# Autodesk Inventor assembly: RCUAssy
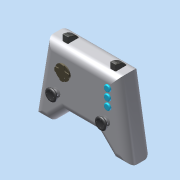
[picture p0: Inventor's stored thumbnail of the model, 180x180]
Saved by Autodesk Inventor 2011 SP1 (Build 150282100, 282)
## iProperties
Created: 2011-08-15
Part Number: RCUAssy
Document SubType Name: Assembly
Designer: dgitz
Author: dgitz
## Documents named in this file (6)
- C:\Dropbox\ICARUS\Remote Control Unit (RCU)\RCU v2\Design\RCUv2-2\RCUAssy.iam
- C:\Dropbox\ICARUS\Remote Control Unit (RCU)\RCU v2\Design\RCUv2-2\RUCBase.ipt
- C:\Dropbox\ICARUS\Remote Control Unit (RCU)\RCU v2\Design\Library\Trigger.ipt
- C:\Dropbox\ICARUS\Remote Control Unit (RCU)\RCU v2\Design\Imported Components\User Library-Joystick_Asm_Left\Assembly3.iam
- C:\Dropbox\ICARUS\Remote Control Unit (RCU)\RCU v2\Design\Library\Xbox360Button.ipt
- C:\Dropbox\ICARUS\Remote Control Unit (RCU)\RCU v2\Design\Library\XBox360DirectionalPad.ipt
## Components (9 placed, 5 different names)
1. RUCBase:1 — Mate:1, Mate:2, Mate:4, Mate:8, Mate:9
2. Trigger:1 — Insert:1, Flush:4, Mate:9
3. Trigger:2 — Insert:1, Flush:4
4. Assembly3:1 [sub-assembly] — Mate:1, Flush:1, Mate:3
5. Assembly3:2 [sub-assembly] — Mate:2, Flush:1, Mate:3
6. XBox360DirectionalPad:1 — Mate:4, Mate:5
7. Xbox360Button:2 — Mate:6, Mate:7, Flush:2, Flush:3
8. Xbox360Button:3 — Mate:7, Flush:3, Mate:8
9. Xbox360Button:4 — Mate:6, Flush:2
## Relationships (14: Mate 9, Flush 4, Insert 1)
- Mate:1 (-6.35 mm): RUCBase:1 ↔ Assembly3:1
- Mate:2 (-6.35 mm): RUCBase:1 ↔ Assembly3:2
- Flush:1: Assembly3:1 ↔ Assembly3:2
- Mate:3 (63.5 mm): Assembly3:1 ↔ Assembly3:2
- Insert:1 (76.2 mm): Trigger:1 ↔ Trigger:2
- Mate:4 (-2.54 mm): RUCBase:1 ↔ XBox360DirectionalPad:1
- Mate:5 (-31.75 mm): XBox360DirectionalPad:1
- Mate:6 (12.7 mm): Xbox360Button:2 ↔ Xbox360Button:4
- Mate:7 (12.7 mm): Xbox360Button:2 ↔ Xbox360Button:3
- Flush:2: Xbox360Button:2 ↔ Xbox360Button:4
- Flush:3: Xbox360Button:2 ↔ Xbox360Button:3
- Mate:8 (-15.24 mm): RUCBase:1 ↔ Xbox360Button:3
- Flush:4: Trigger:1 ↔ Trigger:2
- Mate:9: RUCBase:1 ↔ Trigger:1
